# Autodesk Inventor assembly: Camera
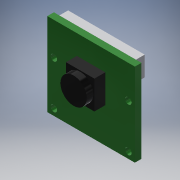
[picture p0: Inventor's stored thumbnail of the model, 180x180]
Saved by Autodesk Inventor 2018 (Build 220112000, 112)
## iProperties
Created: 2018-01-13
Part Number: Camera
Document SubType Name: Assembly
Designer: Kyle-HP
Author: Kyle-HP
## Documents named in this file (4)
- C:\Users\Kyle-HP\Documents\Hackathon-2018\Inventor\Robot\Camera.iam
- C:\Users\Kyle-HP\Documents\Hackathon-2018\Inventor\Robot\CameraBoard.ipt
- C:\Users\Kyle-HP\Documents\Hackathon-2018\Inventor\Robot\CameraLens.ipt
- C:\Users\Kyle-HP\Documents\Hackathon-2018\Inventor\Robot\CameraPlug.ipt
## Components (3 placed, 3 different names)
1. CameraBoard:1 — Mate:1, Flush:1, Flush:2, Mate:2, Flush:3, Flush:4
2. CameraLens:1 — Mate:2, Flush:3, Flush:4
3. CameraPlug:1 — Mate:1, Flush:1, Flush:2
## Relationships (6: Flush 4, Mate 2)
- Mate:1: CameraBoard:1 ↔ CameraPlug:1
- Flush:1: CameraBoard:1 ↔ CameraPlug:1
- Flush:2 (1.5875 mm): CameraBoard:1 ↔ CameraPlug:1
- Mate:2: CameraBoard:1 ↔ CameraLens:1
- Flush:3 (-8.5725 mm): CameraBoard:1 ↔ CameraLens:1
- Flush:4 (5.715 mm): CameraBoard:1 ↔ CameraLens:1
